# Autodesk Inventor assembly: Base
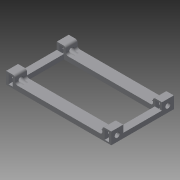
[picture p0: Inventor's stored thumbnail of the model, 180x180]
Saved by Autodesk Inventor 2014 SP1 (Build 180222100, 222)
## iProperties
Created: 2017-05-21
Part Number: Base
Document SubType Name: Assembly
Designer: danielsikar
Author: danielsikar
## Documents named in this file (3)
- C:\Users\danielsikar\Documents\Inventor\FlaskCradle\assemblies\Base.iam
- C:\Users\danielsikar\Documents\Inventor\FlaskCradle\parts\BaseSlat.ipt
- C:\Users\danielsikar\Documents\Inventor\FlaskCradle\parts\CrossBeam2.ipt
## Components (3 placed, 2 different names)
1. BaseSlat:1 — Mate:1, Mate:3, Mate:5, Flush:1, Flush:2
2. BaseSlat:2 — Mate:2, Mate:4, Mate:6, Mate:7
3. CrossBeam2:1 — Flush:1, Flush:2
## Relationships (9: Mate 7, Flush 2)
- Mate:1: BaseSlat:1
- Mate:2: BaseSlat:2
- Mate:3: BaseSlat:1
- Mate:4: BaseSlat:2
- Mate:5: BaseSlat:1
- Mate:6: BaseSlat:2
- Mate:7 (42.5 mm): BaseSlat:2
- Flush:1: BaseSlat:1 ↔ CrossBeam2:1
- Flush:2: BaseSlat:1 ↔ CrossBeam2:1
